# Autodesk Inventor assembly: Accumulator
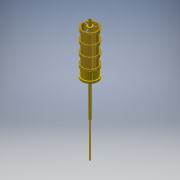
[picture p0: Inventor's stored thumbnail of the model, 180x180]
Saved by Autodesk Inventor 2017 (Build 210142000, 142)
## iProperties
Created: 2009-05-07
Part Number: Accumulator
Document SubType Name: Assembly
Designer: Serena
Author: Serena
## Documents named in this file (10)
- E:\Vault\Designs\Positrons\Accumulator\Accumulator Penning Trap\Acc_PenningTrap.iam
- E:\Vault\Designs\Positrons\Accumulator\Accumulator Penning Trap\Electrode 1.ipt
- E:\Vault\Designs\Positrons\Accumulator\Accumulator Penning Trap\Electrode 2v2.ipt
- E:\Vault\Designs\Positrons\Accumulator\Accumulator Penning Trap\sapphire ball.ipt
- E:\Vault\Designs\Positrons\Accumulator\Accumulator Penning Trap\Electrode 3.ipt
- E:\Vault\Designs\Positrons\Accumulator\Accumulator Penning Trap\Plate between E2 and E3.ipt
- E:\Vault\Designs\Positrons\Accumulator\Accumulator Penning Trap\Plate between E3 and E4.ipt
- E:\Vault\Designs\Positrons\Accumulator\Accumulator Penning Trap\Electrode 5_6_7.ipt
- E:\Vault\Designs\Positrons\Accumulator\Accumulator Penning Trap\Electrode 4.ipt
- E:\Vault\Designs\Positrons\Accumulator\Accumulator Penning Trap\ALPHA_001160_Electrode 8.iam
## Components (159 placed, 9 different names)
1. Electrode 1:1 — Mate:1, Mate:2, Mate:3, Mate:4, Mate:5, Mate:6
2. Electrode 2v2:1 — Mate:7, Mate:8, Mate:9, Mate:10, Mate:11, Mate:12, Mate:13, Mate:14, Mate:15
3. sapphire ball:1 — Mate:4
4. sapphire ball:2 — Mate:5, Mate:8
5. sapphire ball:3 — Mate:6
6. sapphire ball:4 — Mate:1
7. sapphire ball:5 — Mate:3, Mate:9
8. sapphire ball:6 — Mate:2, Mate:7
9. sapphire ball:7 — Mate:10, Mate:18
10. sapphire ball:8 — Mate:11
11. sapphire ball:9 — Mate:14, Mate:17
12. sapphire ball:10 — Mate:15
13. sapphire ball:11 — Mate:13, Mate:16
14. sapphire ball:12 — Mate:12
15. Electrode 3:1 — Mate:27, Mate:28, Mate:29, Mate:30, Mate:31, Mate:32, Mate:33, Mate:34, Mate:35, Mate:36, Mate:37, Mate:175
16. Plate between E2 and E3:1 — Mate:16, Mate:17, Mate:18, Mate:19, Mate:20, Mate:21, Mate:22, Mate:23, Mate:24, Mate:25, Mate:26
17. sapphire ball:13 — Mate:22
18. sapphire ball:14 — Mate:19, Mate:29
19. sapphire ball:15 — Mate:20
20. sapphire ball:16 — Mate:21
21. sapphire ball:17 — Mate:25
22. sapphire ball:18 — Mate:26, Mate:27
23. sapphire ball:19 — Mate:24
24. sapphire ball:20 — Mate:23, Mate:28
25. Plate between E3 and E4:1 — Mate:176, Mate:38, Mate:39, Mate:40, Mate:137, Mate:138, Mate:139, Mate:140, Mate:141, Mate:142, Mate:143, Mate:144, Mate:145, Mate:146, Mate:147, Mate:148, Mate:149, Mate:150, Mate:151, Mate:152, Mate:153, Mate:154, Mate:155, Mate:156, Mate:157, Mate:158, Mate:159, Mate:160, Mate:161, Mate:162, Mate:163, Mate:164, Mate:165, Mate:166, Mate:175
26. sapphire ball:21 — Mate:37
27. sapphire ball:22 — Mate:36, Mate:40
28. sapphire ball:23 — Mate:35
29. sapphire ball:24 — Mate:34, Mate:39
30. sapphire ball:25 — Mate:33
31. sapphire ball:26 — Mate:32, Mate:38
32. sapphire ball:27 — Mate:31
33. sapphire ball:28 — Mate:30
34. Electrode 5_6_7:1 — Mate:41, Mate:42, Mate:43, Mate:44, Mate:45, Mate:46, Mate:47, Mate:48, Mate:49, Mate:50, Mate:51, Mate:52, Mate:53, Mate:54, Mate:55, Mate:56, Mate:57, Mate:58, Mate:59, Mate:60, Mate:61, Mate:62, Mate:63, Mate:64, Mate:65, Mate:66, Mate:67, Mate:68, Mate:69, Mate:70, Mate:71, Mate:72, Mate:73, Mate:74, Mate:75, Mate:76, Mate:77, Mate:78, Mate:79, Mate:80, Mate:81, Mate:82, Mate:83, Mate:84, Mate:85, Mate:86, Mate:87, Mate:88, Mate:89, Mate:90, Mate:91, Mate:92, Mate:93, Mate:94, Mate:95, Mate:96, Mate:97, Mate:98, Mate:99, Mate:100, Mate:176, Mate:177
35. Electrode 5_6_7:2 — Mate:134, Mate:135, Mate:136, Mate:173, Mate:174
36. Electrode 5_6_7:3 — Mate:101, Mate:102, Mate:103, Mate:104, Mate:105, Mate:106, Mate:107, Mate:108, Mate:109, Mate:110, Mate:111, Mate:112, Mate:113, Mate:114, Mate:115, Mate:116, Mate:117, Mate:118, Mate:119, Mate:120, Mate:121, Mate:122, Mate:123, Mate:124, Mate:125, Mate:126, Mate:127, Mate:128, Mate:129, Mate:130, Mate:131, Mate:132, Mate:133
37. sapphire ball:29 — Mate:43
38. sapphire ball:30 — Mate:44
39. sapphire ball:31 — Mate:45
40. sapphire ball:32 — Mate:46
41. sapphire ball:33 — Mate:47
42. sapphire ball:34 — Mate:48
43. sapphire ball:35 — Mate:49
44. sapphire ball:36 — Mate:50, Tangent:1
45. sapphire ball:37 — Mate:51
46. sapphire ball:38 — Mate:52
47. sapphire ball:39 — Mate:53
48. sapphire ball:40 — Mate:54
49. sapphire ball:41 — Mate:55
50. sapphire ball:42 — Mate:56
51. sapphire ball:43 — Mate:57
52. sapphire ball:44 — Mate:58
53. sapphire ball:45 — Mate:59
54. sapphire ball:46 — Mate:60
55. sapphire ball:47 — Mate:61
56. sapphire ball:48 — Mate:62
57. sapphire ball:49 — Mate:63
58. sapphire ball:50 — Mate:64
59. sapphire ball:51 — Mate:65
60. sapphire ball:52 — Mate:66
61. sapphire ball:53 — Mate:67
62. sapphire ball:54 — Mate:68
63. sapphire ball:55 — Mate:69
64. sapphire ball:56 — Mate:70
65. sapphire ball:57 — Mate:41
66. sapphire ball:58 — Mate:42
67. sapphire ball:59 — Mate:71
68. sapphire ball:60 — Mate:100
69. sapphire ball:61 — Mate:99
70. sapphire ball:62 — Mate:98
71. sapphire ball:63 — Mate:97
72. sapphire ball:64 — Mate:96
73. sapphire ball:65 — Mate:95
74. sapphire ball:66 — Mate:94
75. sapphire ball:67 — Mate:93
76. sapphire ball:68 — Mate:92
77. sapphire ball:69 — Mate:91
78. sapphire ball:70 — Mate:90
79. sapphire ball:71 — Mate:89
80. sapphire ball:72 — Mate:88
81. sapphire ball:73 — Mate:87
82. sapphire ball:74 — Mate:86
83. sapphire ball:75 — Mate:85
84. sapphire ball:76 — Mate:84
85. sapphire ball:77 — Mate:83
86. sapphire ball:78 — Mate:82
87. sapphire ball:79 — Mate:81
88. sapphire ball:80 — Mate:80
89. sapphire ball:81 — Mate:79
90. sapphire ball:82 — Mate:78
91. sapphire ball:83 — Mate:77
92. sapphire ball:84 — Mate:76, Mate:103
93. sapphire ball:85 — Mate:75
94. sapphire ball:86 — Mate:74, Mate:102
95. sapphire ball:87 — Mate:73
96. sapphire ball:88 — Mate:72, Mate:101
97. sapphire ball:89 — Mate:105, Mate:135
98. sapphire ball:90 — Mate:104
99. sapphire ball:91 — Mate:133, Mate:136
100. sapphire ball:92 — Mate:132
101. sapphire ball:93 — Mate:131
102. sapphire ball:94 — Mate:130
103. sapphire ball:95 — Mate:129
104. sapphire ball:96 — Mate:128
105. sapphire ball:97 — Mate:127
106. sapphire ball:98 — Mate:126
107. sapphire ball:99 — Mate:125
108. sapphire ball:100 — Mate:124
109. sapphire ball:101 — Mate:123
110. sapphire ball:102 — Mate:122
111. sapphire ball:103 — Mate:121
112. sapphire ball:104 — Mate:120
113. sapphire ball:105 — Mate:119
114. sapphire ball:106 — Mate:118
115. sapphire ball:107 — Mate:117
116. sapphire ball:108 — Mate:116
117. sapphire ball:109 — Mate:115
118. sapphire ball:110 — Mate:114
119. sapphire ball:111 — Mate:113
120. sapphire ball:112 — Mate:112
121. sapphire ball:113 — Mate:111
122. sapphire ball:114 — Mate:110
123. sapphire ball:115 — Mate:109
124. sapphire ball:116 — Mate:108
125. sapphire ball:117 — Mate:107, Mate:134
126. sapphire ball:118 — Mate:106
127. Electrode 4:1 — Mate:177, Tangent:1, Tangent:2
128. sapphire ball:119 — Mate:166
129. sapphire ball:120 — Mate:164
130. sapphire ball:121 — Mate:165, Tangent:2
131. sapphire ball:122 — Mate:162
132. sapphire ball:123 — Mate:163
133. sapphire ball:124 — Mate:161
134. sapphire ball:125 — Mate:160
135. sapphire ball:126 — Mate:159
136. sapphire ball:127 — Mate:139
137. sapphire ball:128 — Mate:137
138. sapphire ball:129 — Mate:138
139. sapphire ball:130 — Mate:140
140. sapphire ball:131 — Mate:141
141. sapphire ball:132 — Mate:142
142. sapphire ball:133 — Mate:143
143. sapphire ball:134 — Mate:144
144. sapphire ball:135 — Mate:145
145. sapphire ball:136 — Mate:146
146. sapphire ball:137 — Mate:147
147. sapphire ball:138 — Mate:148
148. sapphire ball:139 — Mate:149
149. sapphire ball:140 — Mate:150
150. sapphire ball:141 — Mate:151
151. sapphire ball:142 — Mate:152
152. sapphire ball:143 — Mate:153
153. sapphire ball:144 — Mate:154
154. sapphire ball:145 — Mate:155
155. sapphire ball:146 — Mate:156
156. sapphire ball:147 — Mate:157
157. sapphire ball:148 — Mate:158
158. ALPHA_001160_Electrode 8:1 [sub-assembly] — Mate:173, Mate:174
159. sapphire ball:149
## Relationships (173: Mate 171, Tangent 2)
- Mate:1: Electrode 1:1 ↔ sapphire ball:4
- Mate:2: Electrode 1:1 ↔ sapphire ball:6
- Mate:3: Electrode 1:1 ↔ sapphire ball:5
- Mate:4: Electrode 1:1 ↔ sapphire ball:1
- Mate:5: Electrode 1:1 ↔ sapphire ball:2
- Mate:6: Electrode 1:1 ↔ sapphire ball:3
- Mate:7: Electrode 2v2:1 ↔ sapphire ball:6
- Mate:8: Electrode 2v2:1 ↔ sapphire ball:2
- Mate:9: Electrode 2v2:1 ↔ sapphire ball:5
- Mate:10: Electrode 2v2:1 ↔ sapphire ball:7
- Mate:11: Electrode 2v2:1 ↔ sapphire ball:8
- Mate:12: Electrode 2v2:1 ↔ sapphire ball:12
- Mate:13: Electrode 2v2:1 ↔ sapphire ball:11
- Mate:14: Electrode 2v2:1 ↔ sapphire ball:9
- Mate:15: Electrode 2v2:1 ↔ sapphire ball:10
- Mate:16: sapphire ball:11 ↔ Plate between E2 and E3:1
- Mate:17: sapphire ball:9 ↔ Plate between E2 and E3:1
- Mate:18: sapphire ball:7 ↔ Plate between E2 and E3:1
- Mate:19: Plate between E2 and E3:1 ↔ sapphire ball:14
- Mate:20: Plate between E2 and E3:1 ↔ sapphire ball:15
- Mate:21: Plate between E2 and E3:1 ↔ sapphire ball:16
- Mate:22: Plate between E2 and E3:1 ↔ sapphire ball:13
- Mate:23: Plate between E2 and E3:1 ↔ sapphire ball:20
- Mate:24: Plate between E2 and E3:1 ↔ sapphire ball:19
- Mate:25: Plate between E2 and E3:1 ↔ sapphire ball:17
- Mate:26: Plate between E2 and E3:1 ↔ sapphire ball:18
- Mate:27: Electrode 3:1 ↔ sapphire ball:18
- Mate:28: Electrode 3:1 ↔ sapphire ball:20
- Mate:29: Electrode 3:1 ↔ sapphire ball:14
- Mate:30: Electrode 3:1 ↔ sapphire ball:28
- Mate:31: Electrode 3:1 ↔ sapphire ball:27
- Mate:32: Electrode 3:1 ↔ sapphire ball:26
- Mate:33: Electrode 3:1 ↔ sapphire ball:25
- Mate:34: Electrode 3:1 ↔ sapphire ball:24
- Mate:35: Electrode 3:1 ↔ sapphire ball:23
- Mate:36: Electrode 3:1 ↔ sapphire ball:22
- Mate:37: Electrode 3:1 ↔ sapphire ball:21
- Mate:176: Plate between E3 and E4:1 ↔ Electrode 5_6_7:1
- Mate:38: Plate between E3 and E4:1 ↔ sapphire ball:26
- Mate:39: Plate between E3 and E4:1 ↔ sapphire ball:24
- Mate:40: Plate between E3 and E4:1 ↔ sapphire ball:22
- Mate:41: Electrode 5_6_7:1 ↔ sapphire ball:57
- Mate:42: Electrode 5_6_7:1 ↔ sapphire ball:58
- Mate:43: Electrode 5_6_7:1 ↔ sapphire ball:29
- Mate:44: Electrode 5_6_7:1 ↔ sapphire ball:30
- Mate:45: Electrode 5_6_7:1 ↔ sapphire ball:31
- Mate:46: Electrode 5_6_7:1 ↔ sapphire ball:32
- Mate:47: Electrode 5_6_7:1 ↔ sapphire ball:33
- Mate:48: Electrode 5_6_7:1 ↔ sapphire ball:34
- Mate:49: Electrode 5_6_7:1 ↔ sapphire ball:35
- Mate:50: Electrode 5_6_7:1 ↔ sapphire ball:36
- Mate:51: Electrode 5_6_7:1 ↔ sapphire ball:37
- Mate:52: Electrode 5_6_7:1 ↔ sapphire ball:38
- Mate:53: Electrode 5_6_7:1 ↔ sapphire ball:39
- Mate:54: Electrode 5_6_7:1 ↔ sapphire ball:40
- Mate:55: Electrode 5_6_7:1 ↔ sapphire ball:41
- Mate:56: Electrode 5_6_7:1 ↔ sapphire ball:42
- Mate:57: Electrode 5_6_7:1 ↔ sapphire ball:43
- Mate:58: Electrode 5_6_7:1 ↔ sapphire ball:44
- Mate:59: Electrode 5_6_7:1 ↔ sapphire ball:45
- Mate:60: Electrode 5_6_7:1 ↔ sapphire ball:46
- Mate:61: Electrode 5_6_7:1 ↔ sapphire ball:47
- Mate:62: Electrode 5_6_7:1 ↔ sapphire ball:48
- Mate:63: Electrode 5_6_7:1 ↔ sapphire ball:49
- Mate:64: Electrode 5_6_7:1 ↔ sapphire ball:50
- Mate:65: Electrode 5_6_7:1 ↔ sapphire ball:51
- Mate:66: Electrode 5_6_7:1 ↔ sapphire ball:52
- Mate:67: Electrode 5_6_7:1 ↔ sapphire ball:53
- Mate:68: Electrode 5_6_7:1 ↔ sapphire ball:54
- Mate:69: Electrode 5_6_7:1 ↔ sapphire ball:55
- Mate:70: Electrode 5_6_7:1 ↔ sapphire ball:56
- Mate:71: Electrode 5_6_7:1 ↔ sapphire ball:59
- Mate:72: Electrode 5_6_7:1 ↔ sapphire ball:88
- Mate:73: Electrode 5_6_7:1 ↔ sapphire ball:87
- Mate:74: Electrode 5_6_7:1 ↔ sapphire ball:86
- Mate:75: Electrode 5_6_7:1 ↔ sapphire ball:85
- Mate:76: Electrode 5_6_7:1 ↔ sapphire ball:84
- Mate:77: Electrode 5_6_7:1 ↔ sapphire ball:83
- Mate:78: Electrode 5_6_7:1 ↔ sapphire ball:82
- Mate:79: Electrode 5_6_7:1 ↔ sapphire ball:81
- Mate:80: Electrode 5_6_7:1 ↔ sapphire ball:80
- Mate:81: Electrode 5_6_7:1 ↔ sapphire ball:79
- Mate:82: Electrode 5_6_7:1 ↔ sapphire ball:78
- Mate:83: Electrode 5_6_7:1 ↔ sapphire ball:77
- Mate:84: Electrode 5_6_7:1 ↔ sapphire ball:76
- Mate:85: Electrode 5_6_7:1 ↔ sapphire ball:75
- Mate:86: Electrode 5_6_7:1 ↔ sapphire ball:74
- Mate:87: Electrode 5_6_7:1 ↔ sapphire ball:73
- Mate:88: Electrode 5_6_7:1 ↔ sapphire ball:72
- Mate:89: Electrode 5_6_7:1 ↔ sapphire ball:71
- Mate:90: Electrode 5_6_7:1 ↔ sapphire ball:70
- Mate:91: Electrode 5_6_7:1 ↔ sapphire ball:69
- Mate:92: Electrode 5_6_7:1 ↔ sapphire ball:68
- Mate:93: Electrode 5_6_7:1 ↔ sapphire ball:67
- Mate:94: Electrode 5_6_7:1 ↔ sapphire ball:66
- Mate:95: Electrode 5_6_7:1 ↔ sapphire ball:65
- Mate:96: Electrode 5_6_7:1 ↔ sapphire ball:64
- Mate:97: Electrode 5_6_7:1 ↔ sapphire ball:63
- Mate:98: Electrode 5_6_7:1 ↔ sapphire ball:62
- Mate:99: Electrode 5_6_7:1 ↔ sapphire ball:61
- Mate:100: Electrode 5_6_7:1 ↔ sapphire ball:60
- Mate:101: Electrode 5_6_7:3 ↔ sapphire ball:88
- Mate:102: Electrode 5_6_7:3 ↔ sapphire ball:86
- Mate:103: Electrode 5_6_7:3 ↔ sapphire ball:84
- Mate:104: Electrode 5_6_7:3 ↔ sapphire ball:90
- Mate:105: Electrode 5_6_7:3 ↔ sapphire ball:89
- Mate:106: Electrode 5_6_7:3 ↔ sapphire ball:118
- Mate:107: Electrode 5_6_7:3 ↔ sapphire ball:117
- Mate:108: Electrode 5_6_7:3 ↔ sapphire ball:116
- Mate:109: Electrode 5_6_7:3 ↔ sapphire ball:115
- Mate:110: Electrode 5_6_7:3 ↔ sapphire ball:114
- Mate:111: Electrode 5_6_7:3 ↔ sapphire ball:113
- Mate:112: Electrode 5_6_7:3 ↔ sapphire ball:112
- Mate:113: Electrode 5_6_7:3 ↔ sapphire ball:111
- Mate:114: Electrode 5_6_7:3 ↔ sapphire ball:110
- Mate:115: Electrode 5_6_7:3 ↔ sapphire ball:109
- Mate:116: Electrode 5_6_7:3 ↔ sapphire ball:108
- Mate:117: Electrode 5_6_7:3 ↔ sapphire ball:107
- Mate:118: Electrode 5_6_7:3 ↔ sapphire ball:106
- Mate:119: Electrode 5_6_7:3 ↔ sapphire ball:105
- Mate:120: Electrode 5_6_7:3 ↔ sapphire ball:104
- Mate:121: Electrode 5_6_7:3 ↔ sapphire ball:103
- Mate:122: Electrode 5_6_7:3 ↔ sapphire ball:102
- Mate:123: Electrode 5_6_7:3 ↔ sapphire ball:101
- Mate:124: Electrode 5_6_7:3 ↔ sapphire ball:100
- Mate:125: Electrode 5_6_7:3 ↔ sapphire ball:99
- Mate:126: Electrode 5_6_7:3 ↔ sapphire ball:98
- Mate:127: Electrode 5_6_7:3 ↔ sapphire ball:97
- Mate:128: Electrode 5_6_7:3 ↔ sapphire ball:96
- Mate:129: Electrode 5_6_7:3 ↔ sapphire ball:95
- Mate:130: Electrode 5_6_7:3 ↔ sapphire ball:94
- Mate:131: Electrode 5_6_7:3 ↔ sapphire ball:93
- Mate:132: Electrode 5_6_7:3 ↔ sapphire ball:92
- Mate:133: Electrode 5_6_7:3 ↔ sapphire ball:91
- Mate:134: Electrode 5_6_7:2 ↔ sapphire ball:117
- Mate:135: Electrode 5_6_7:2 ↔ sapphire ball:89
- Mate:136: Electrode 5_6_7:2 ↔ sapphire ball:91
- Mate:137: Plate between E3 and E4:1 ↔ sapphire ball:128
- Mate:138: Plate between E3 and E4:1 ↔ sapphire ball:129
- Mate:139: Plate between E3 and E4:1 ↔ sapphire ball:127
- Mate:140: Plate between E3 and E4:1 ↔ sapphire ball:130
- Mate:141: Plate between E3 and E4:1 ↔ sapphire ball:131
- Mate:142: Plate between E3 and E4:1 ↔ sapphire ball:132
- Mate:143: Plate between E3 and E4:1 ↔ sapphire ball:133
- Mate:144: Plate between E3 and E4:1 ↔ sapphire ball:134
- Mate:145: Plate between E3 and E4:1 ↔ sapphire ball:135
- Mate:146: Plate between E3 and E4:1 ↔ sapphire ball:136
- Mate:147: Plate between E3 and E4:1 ↔ sapphire ball:137
- Mate:148: Plate between E3 and E4:1 ↔ sapphire ball:138
- Mate:149: Plate between E3 and E4:1 ↔ sapphire ball:139
- Mate:150: Plate between E3 and E4:1 ↔ sapphire ball:140
- Mate:151: Plate between E3 and E4:1 ↔ sapphire ball:141
- Mate:152: Plate between E3 and E4:1 ↔ sapphire ball:142
- Mate:153: Plate between E3 and E4:1 ↔ sapphire ball:143
- Mate:154: Plate between E3 and E4:1 ↔ sapphire ball:144
- Mate:155: Plate between E3 and E4:1 ↔ sapphire ball:145
- Mate:156: Plate between E3 and E4:1 ↔ sapphire ball:146
- Mate:157: Plate between E3 and E4:1 ↔ sapphire ball:147
- Mate:158: Plate between E3 and E4:1 ↔ sapphire ball:148
- Mate:159: Plate between E3 and E4:1 ↔ sapphire ball:126
- Mate:160: Plate between E3 and E4:1 ↔ sapphire ball:125
- Mate:161: Plate between E3 and E4:1 ↔ sapphire ball:124
- Mate:162: Plate between E3 and E4:1 ↔ sapphire ball:122
- Mate:163: Plate between E3 and E4:1 ↔ sapphire ball:123
- Mate:164: Plate between E3 and E4:1 ↔ sapphire ball:120
- Mate:165: Plate between E3 and E4:1 ↔ sapphire ball:121
- Mate:166: Plate between E3 and E4:1 ↔ sapphire ball:119
- Mate:173 (0.762 mm): Electrode 5_6_7:2 ↔ ALPHA_001160_Electrode 8:1
- Mate:174: Electrode 5_6_7:2 ↔ ALPHA_001160_Electrode 8:1
- Mate:175: Electrode 3:1 ↔ Plate between E3 and E4:1
- Mate:177: Electrode 5_6_7:1 ↔ Electrode 4:1
- Tangent:1: sapphire ball:36 ↔ Electrode 4:1
- Tangent:2: Electrode 4:1 ↔ sapphire ball:121
